# Autodesk Inventor assembly: PumpeV1
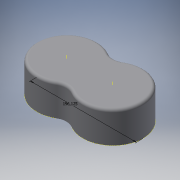
[picture p0: Inventor's stored thumbnail of the model, 180x180]
Saved by Autodesk Inventor 2017 (Build 210142000, 142)
## iProperties
Created: 2019-05-23
Part Number: PumpeV1
Document SubType Name: Assembly
Designer: Ole Simmering
Author: Ole Simmering
## Documents named in this file (3)
- C:\Users\Ole Simmering\Documents\3d modelling fun\HA4-Zahnradpumpe\PumpeV1.iam
- C:\Users\Ole Simmering\Documents\3d modelling fun\HA4-Zahnradpumpe\Gehaeuse_V2.ipt
- C:\Users\Ole Simmering\Documents\3d modelling fun\HA4-Zahnradpumpe\Zahnrad95x50.ipt
## Components (3 placed, 2 different names)
1. Gehaeuse_V2:1 — Mate:1, Mate:2, Mate:3, Mate:4
2. Zahnrad95x50:1 — Mate:1, Mate:2
3. Zahnrad95x50:2 — Mate:3, Mate:4
## Relationships (4: Mate 4)
- Mate:1: Gehaeuse_V2:1 ↔ Zahnrad95x50:1
- Mate:2: Gehaeuse_V2:1 ↔ Zahnrad95x50:1
- Mate:3: Gehaeuse_V2:1 ↔ Zahnrad95x50:2
- Mate:4: Gehaeuse_V2:1 ↔ Zahnrad95x50:2
